# Autodesk Inventor assembly: Main Assembly
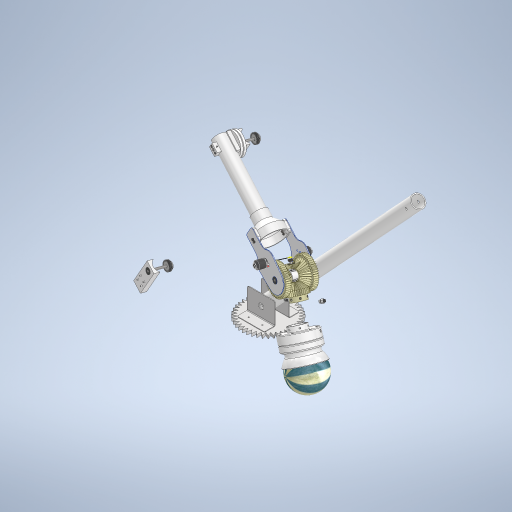
[picture p0: Inventor's stored thumbnail of the model, 512x512]
Saved by Autodesk Inventor 2023 (Build 270158030, 158C)
## iProperties
Created: 2022-10-01
Part Number: Main Assembly
Document SubType Name: Assembly
Designer: cjj5381
Mass: 5062.37 g
Surface Area: 13451.6 cm^2
Volume: 4101.5 cm^3
Density: 1.23427 g/cm^3
Author: cjj5381
## Documents named in this file (21)
- V:\Robtotics\Main Assembly.iam
- V:\Robtotics\Arm Segment 1.ipt
- V:\Robtotics\3 Stage HD - CIM Sport.iam
- V:\Robtotics\am-4259 NEO 550 Brushless Motor.ipt
- V:\Robtotics\Arm Segment 2.ipt
- V:\Robtotics\Wrist\Wrist.iam
- V:\Robtotics\Versaball.iam
- V:\Robtotics\Hardware\91290A224_NO THREADS_Alloy Steel Socket Head Screw.ipt
- V:\Robtotics\Hardware\7397N19_NO THREADS_Universal-Thread Push-to-Connect Tube Fittings.ipt
- V:\Robtotics\Hub Plate.ipt
- V:\Robtotics\Hardware\5909K15_Needle-Roller Thrust Bearing.ipt
- V:\Robtotics\Hardware\5909K75_1 mm Thick Washer for 20 mm Shaft Diameter Needle-Roller Thrust Bearing.ipt
- V:\Robtotics\Motor Mount.ipt
- V:\Robtotics\Hardware\91251A342_NO THREADS_Black-Oxide Alloy Steel Socket Head Screw.ipt
- V:\Robtotics\Hardware\1265K77_Rotary Shaft-longer.ipt
- V:\Robtotics\Axial Holder.ipt
- V:\Robtotics\Hardware\91290A254_NO THREADS_Black-Oxide Alloy Steel Socket Head Screw.ipt
- V:\Robtotics\Hardware\GPA60GT2060-B-NK10.iam
- V:\Robtotics\Hardware\2349K412_Permanently Lubricated Ball Bearing.ipt
- V:\Robtotics\Hardware\1265K77_Rotary Shaft short.ipt
- V:\Robtotics\Base\Base.iam
## Components (35 placed, 20 different names)
1. Base:1 [sub-assembly] — Mate:1, Flush:1, Mate:2, Mate:3
2. Arm Segment 1:1 — Mate:2, Mate:3
3. 3 Stage HD - CIM Sport:2 [sub-assembly]
4. am-4259 NEO 550 Brushless Motor:1
5. am-4259 NEO 550 Brushless Motor:2
6. Arm Segment 2:1
7. Wrist:1 [sub-assembly]
8. Versaball:1 [sub-assembly]
9. 7397N19_NO THREADS_Universal-Thread Push-to-Connect Tube Fittings:1
10. Hub Plate:1
11. Hub Plate:2
12. 5909K15_Needle-Roller Thrust Bearing:1
13. 5909K75_1 mm Thick Washer for 20 mm Shaft Diameter Needle-Roller Thrust Bearing:1
14. 5909K75_1 mm Thick Washer for 20 mm Shaft Diameter Needle-Roller Thrust Bearing:2
15. Motor Mount:1
16. 1265K77_Rotary Shaft-longer:1
17. Axial Holder:1
18. 91290A254_NO THREADS_Black-Oxide Alloy Steel Socket Head Screw:1
19. 91290A254_NO THREADS_Black-Oxide Alloy Steel Socket Head Screw:2
20. 91290A254_NO THREADS_Black-Oxide Alloy Steel Socket Head Screw:3
21. GPA60GT2060-B-NK10:1 [sub-assembly]
22. GPA60GT2060-B-NK10:2 [sub-assembly]
23. 2349K412_Permanently Lubricated Ball Bearing:1
24. 1265K77_Rotary Shaft short:1
25. 3 Stage HD - CIM Sport:3 [sub-assembly]
26. 91290A224_NO THREADS_Alloy Steel Socket Head Screw:1
27. 91290A224_NO THREADS_Alloy Steel Socket Head Screw:2
28. 91290A224_NO THREADS_Alloy Steel Socket Head Screw:3
29. 91290A224_NO THREADS_Alloy Steel Socket Head Screw:4
30. 91290A224_NO THREADS_Alloy Steel Socket Head Screw:5
31. 91290A224_NO THREADS_Alloy Steel Socket Head Screw:6
32. 91251A342_NO THREADS_Black-Oxide Alloy Steel Socket Head Screw:1
33. 91251A342_NO THREADS_Black-Oxide Alloy Steel Socket Head Screw:2
34. 91251A342_NO THREADS_Black-Oxide Alloy Steel Socket Head Screw:3
35. 91251A342_NO THREADS_Black-Oxide Alloy Steel Socket Head Screw:4
## Component patterns: (6 elements, first: 91290A224_NO THREADS_Alloy Steel Socket Head Screw:1), (4 elements, first: 91251A342_NO THREADS_Black-Oxide Alloy Steel Socket Head Screw:1)
## Relationships (4: Mate 3, Flush 1)
- Mate:1: Base:1
- Flush:1: Base:1
- Mate:2: Base:1 ↔ Arm Segment 1:1
- Mate:3: Base:1 ↔ Arm Segment 1:1
